# Autodesk Inventor assembly: Cube 1x1 V5 (Camera)
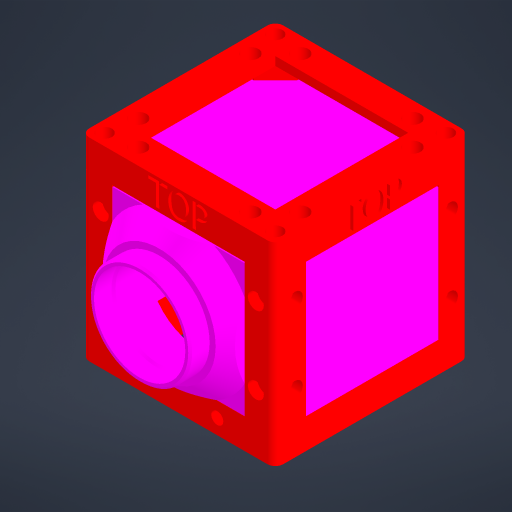
[picture p0: Inventor's stored thumbnail of the model, 512x512]
Saved by Autodesk Inventor 2023.4 (Build 274418000, 418)
## iProperties
Created: 2022-08-13
Part Number: Cube 1x1 V5 (Camera)
Document SubType Name: Assembly
Designer: xSibe
Author: xSibe
## Documents named in this file (4)
- C:\.Laptop\.Work\Projects\Project Protocube\Protocube\CAD, STL, OBJ Files\1 CAD\Camera\Cube 1x1 V5 (Camera).iam
- C:\.Laptop\.Work\Projects\Project Protocube\Protocube\CAD, STL, OBJ Files\1 CAD\Camera\Camera Mount Side.ipt
- C:\.Laptop\.Work\Projects\Project Protocube\Protocube\CAD, STL, OBJ Files\1 CAD\Camera\Camera Mount Adapter.ipt
- C:\.Laptop\.Work\Projects\Project Protocube\Protocube\CAD, STL, OBJ Files\1 CAD\Cubes\Cube 1x1 V5.iam
## Components (3 placed, 3 different names)
1. Camera Mount Side:1 — Mate:1, Mate:3, Mate:4, Mate:5, Mate:6
2. Camera Mount Adapter:1 — Mate:1, Flush:1, Mate:5
3. Cube 1x1 V5:1 [sub-assembly] — Mate:6
## Relationships (6: Mate 5, Flush 1)
- Mate:1: Camera Mount Side:1 ↔ Camera Mount Adapter:1
- Flush:1: Camera Mount Adapter:1
- Mate:3: Camera Mount Side:1
- Mate:4: Camera Mount Side:1
- Mate:5: Camera Mount Side:1 ↔ Camera Mount Adapter:1
- Mate:6: Camera Mount Side:1 ↔ Cube 1x1 V5:1
